# Autodesk Inventor assembly: Car Assembly - Solo
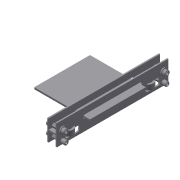
[picture p0: Inventor's stored thumbnail of the model, 180x180]
Saved by Autodesk Inventor 2015 (Build 190159000, 159)
## iProperties
Created: 2014-07-18
Part Number: Car Assembly - Solo
Document SubType Name: Assembly
Designer: Owner
Author: Owner
## Documents named in this file (9)
- T:\FILES\Inventor 2015 Projects\Elevator Version 2\Frc Chassis 2014\Car Assembly - Solo.iam
- T:\FILES\Inventor 2015 Projects\Elevator Version 2\Frc Chassis 2014\car frame.ipt
- T:\FILES\Inventor 2015 Projects\Elevator Version 2\Frc Chassis 2014\#8 .5 Hex Standoff.ipt
- T:\FILES\Inventor 2015 Projects\Elevator Version 2\Frc Chassis 2014\.25 #8 .3125 Spacer.ipt
- T:\FILES\Inventor 2015 Projects\Elevator Version 2\Frc Chassis 2014\Flange Sleve Bearing .25.375 .ipt
- T:\FILES\Inventor 2015 Projects\Elevator Version 2\Frc Chassis 2014\Sleeve Bearing .25 .3125 .ipt
- T:\FILES\Inventor 2015 Projects\Elevator Version 2\Frc Chassis 2014\.375 .75 .375 Nylon Spacer.ipt
- T:\FILES\Inventor 2015 Projects\Elevator Version 2\Frc Chassis 2014\.25 #8 .5625 Spacer.ipt
- T:\FILES\Inventor 2015 Projects\Elevator Version 2\Frc Chassis 2014\Inter-rail plate.ipt
## Components (30 placed, 8 different names)
1. car frame:1 — Mate:1, Mate:2, Mate:3, Mate:4, Mate:8, Mate:9, Mate:13, Mate:14, Mate:16, Mate:17, Mate:18, Mate:22, Mate:23, Mate:24, Mate:30, Mate:31, Mate:32, Mate:33, Mate:34, Mate:35, Mate:36, Mate:38, Mate:39, Mate:40, Mate:41, Mate:42, Mate:44, Mate:46, Mate:47, Mate:48, Mate:74, Mate:75, Mate:78, Mate:79, Mate:80, Mate:81, Mate:82
2. #8 .5 Hex Standoff:1 — Mate:16, Mate:17
3. #8 .5 Hex Standoff:2 — Mate:1, Mate:2
4. #8 .5 Hex Standoff:3 — Mate:30, Mate:31
5. #8 .5 Hex Standoff:4 — Mate:32, Mate:33
6. .25 #8 .3125 Spacer:1 — Mate:46, Mate:48, Mate:49
7. .25 #8 .3125 Spacer:2 — Mate:34, Mate:35, Mate:37
8. .25 #8 .3125 Spacer:3 — Mate:13, Mate:14, Mate:19
9. .25 #8 .3125 Spacer:4 — Mate:22, Mate:23, Mate:25
10. .25 #8 .3125 Spacer:5 — Mate:8, Mate:9, Flush:2, Mate:10
11. .25 #8 .3125 Spacer:6 — Mate:3, Mate:4, Mate:5, Flush:1
12. .25 #8 .3125 Spacer:7 — Mate:39, Mate:41, Mate:45
13. .25 #8 .3125 Spacer:8 — Mate:38, Mate:40, Mate:43
14. Flange Sleve Bearing .25.375 :1 — Mate:47, Mate:49
15. Flange Sleve Bearing .25.375 :2 — Mate:24, Mate:25
16. Flange Sleve Bearing .25.375 :5 — Mate:44, Mate:45
17. Flange Sleve Bearing .25.375 :6 — Mate:18, Mate:19
18. Sleeve Bearing .25 .3125 :1 — Mate:42, Mate:43
19. Sleeve Bearing .25 .3125 :2 — Mate:36, Mate:37
20. Sleeve Bearing .25 .3125 :3 — Flush:2, Mate:10
21. Sleeve Bearing .25 .3125 :4 — Mate:5, Flush:1
22. .375 .75 .375 Nylon Spacer:1 — Mate:58, Mate:60, Mate:63, Mate:64
23. .375 .75 .375 Nylon Spacer:2 — Mate:59, Mate:61, Mate:62, Mate:65
24. Flange Sleve Bearing .25.375 :7 — Mate:63, Mate:64, Mate:66
25. Flange Sleve Bearing .25.375 :8 — Mate:62, Mate:65, Mate:67
26. Flange Sleve Bearing .25.375 :9 — Mate:58, Mate:60, Mate:69
27. Flange Sleve Bearing .25.375 :10 — Mate:59, Mate:61, Mate:68
28. .25 #8 .5625 Spacer:1 — Mate:66, Mate:69, Mate:75, Mate:82
29. .25 #8 .5625 Spacer:2 — Mate:67, Mate:68, Mate:74, Mate:81
30. Inter-rail plate:1 — Mate:78, Mate:79, Mate:80
## Relationships (59: Mate 57, Flush 2)
- Mate:1: car frame:1 ↔ #8 .5 Hex Standoff:2
- Mate:2: car frame:1 ↔ #8 .5 Hex Standoff:2
- Mate:3: car frame:1 ↔ .25 #8 .3125 Spacer:6
- Mate:4: car frame:1 ↔ .25 #8 .3125 Spacer:6
- Mate:5: .25 #8 .3125 Spacer:6 ↔ Sleeve Bearing .25 .3125 :4
- Flush:1: .25 #8 .3125 Spacer:6 ↔ Sleeve Bearing .25 .3125 :4
- Mate:8: car frame:1 ↔ .25 #8 .3125 Spacer:5
- Mate:9: car frame:1 ↔ .25 #8 .3125 Spacer:5
- Flush:2: .25 #8 .3125 Spacer:5 ↔ Sleeve Bearing .25 .3125 :3
- Mate:10: .25 #8 .3125 Spacer:5 ↔ Sleeve Bearing .25 .3125 :3
- Mate:13: car frame:1 ↔ .25 #8 .3125 Spacer:3
- Mate:14: car frame:1 ↔ .25 #8 .3125 Spacer:3
- Mate:16: car frame:1 ↔ #8 .5 Hex Standoff:1
- Mate:17: car frame:1 ↔ #8 .5 Hex Standoff:1
- Mate:18 (0.635 mm): car frame:1 ↔ Flange Sleve Bearing .25.375 :6
- Mate:19: .25 #8 .3125 Spacer:3 ↔ Flange Sleve Bearing .25.375 :6
- Mate:22: car frame:1 ↔ .25 #8 .3125 Spacer:4
- Mate:23: car frame:1 ↔ .25 #8 .3125 Spacer:4
- Mate:24 (0.635 mm): car frame:1 ↔ Flange Sleve Bearing .25.375 :2
- Mate:25: .25 #8 .3125 Spacer:4 ↔ Flange Sleve Bearing .25.375 :2
- Mate:30: car frame:1 ↔ #8 .5 Hex Standoff:3
- Mate:31: car frame:1 ↔ #8 .5 Hex Standoff:3
- Mate:32: car frame:1 ↔ #8 .5 Hex Standoff:4
- Mate:33: car frame:1 ↔ #8 .5 Hex Standoff:4
- Mate:34: car frame:1 ↔ .25 #8 .3125 Spacer:2
- Mate:35: car frame:1 ↔ .25 #8 .3125 Spacer:2
- Mate:36 (0.635 mm): car frame:1 ↔ Sleeve Bearing .25 .3125 :2
- Mate:37: .25 #8 .3125 Spacer:2 ↔ Sleeve Bearing .25 .3125 :2
- Mate:38: car frame:1 ↔ .25 #8 .3125 Spacer:8
- Mate:39: car frame:1 ↔ .25 #8 .3125 Spacer:7
- Mate:40: car frame:1 ↔ .25 #8 .3125 Spacer:8
- Mate:41: car frame:1 ↔ .25 #8 .3125 Spacer:7
- Mate:42 (0.635 mm): car frame:1 ↔ Sleeve Bearing .25 .3125 :1
- Mate:43: .25 #8 .3125 Spacer:8 ↔ Sleeve Bearing .25 .3125 :1
- Mate:44 (0.635 mm): car frame:1 ↔ Flange Sleve Bearing .25.375 :5
- Mate:45: .25 #8 .3125 Spacer:7 ↔ Flange Sleve Bearing .25.375 :5
- Mate:46: car frame:1 ↔ .25 #8 .3125 Spacer:1
- Mate:47 (0.635 mm): car frame:1 ↔ Flange Sleve Bearing .25.375 :1
- Mate:48: car frame:1 ↔ .25 #8 .3125 Spacer:1
- Mate:49: .25 #8 .3125 Spacer:1 ↔ Flange Sleve Bearing .25.375 :1
- Mate:58: .375 .75 .375 Nylon Spacer:1 ↔ Flange Sleve Bearing .25.375 :9
- Mate:59: .375 .75 .375 Nylon Spacer:2 ↔ Flange Sleve Bearing .25.375 :10
- Mate:60: .375 .75 .375 Nylon Spacer:1 ↔ Flange Sleve Bearing .25.375 :9
- Mate:61: .375 .75 .375 Nylon Spacer:2 ↔ Flange Sleve Bearing .25.375 :10
- Mate:62: .375 .75 .375 Nylon Spacer:2 ↔ Flange Sleve Bearing .25.375 :8
- Mate:63: .375 .75 .375 Nylon Spacer:1 ↔ Flange Sleve Bearing .25.375 :7
- Mate:64: .375 .75 .375 Nylon Spacer:1 ↔ Flange Sleve Bearing .25.375 :7
- Mate:65: .375 .75 .375 Nylon Spacer:2 ↔ Flange Sleve Bearing .25.375 :8
- Mate:66: Flange Sleve Bearing .25.375 :7 ↔ .25 #8 .5625 Spacer:1
- Mate:67: Flange Sleve Bearing .25.375 :8 ↔ .25 #8 .5625 Spacer:2
- Mate:68 (0.635 mm): Flange Sleve Bearing .25.375 :10 ↔ .25 #8 .5625 Spacer:2
- Mate:69 (0.635 mm): Flange Sleve Bearing .25.375 :9 ↔ .25 #8 .5625 Spacer:1
- Mate:74: car frame:1 ↔ .25 #8 .5625 Spacer:2
- Mate:75: car frame:1 ↔ .25 #8 .5625 Spacer:1
- Mate:78: car frame:1 ↔ Inter-rail plate:1
- Mate:79: car frame:1 ↔ Inter-rail plate:1
- Mate:80 (9.525 mm): car frame:1 ↔ Inter-rail plate:1
- Mate:81: car frame:1 ↔ .25 #8 .5625 Spacer:2
- Mate:82: car frame:1 ↔ .25 #8 .5625 Spacer:1
